# Autodesk Inventor assembly: Rear Z Axis
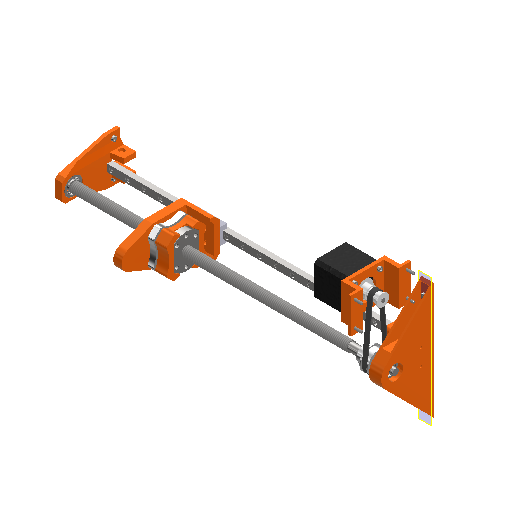
[picture p0: Inventor's stored thumbnail of the model, 512x512]
Saved by Autodesk Inventor 2023.2 (Build 272271000, 271)
## iProperties
Created: 2023-02-15
Part Number: Rear Z Axis
Document SubType Name: Assembly
Designer: remop
Author: remop
## Documents named in this file (20)
- C:\Users\remop\OneDrive\Documents\Inventor\3D Printers\LuEVO\Mk5_FullKinematic\Z Axis v2\Rear\Rear Z Axis.iam
- C:\Users\remop\OneDrive\Documents\Inventor\3D Printers\LuEVO\Mk5_FullKinematic\Z Axis v2\Drivetrain\MGNR9_300mm.ipt
- C:\Users\remop\OneDrive\Documents\Inventor\3D Printers\LuEVO\Mk5_FullKinematic\Z Axis v2\Drivetrain\MGN9H.ipt
- C:\Users\remop\OneDrive\Documents\Inventor\3D Printers\LuEVO\Mk5_FullKinematic\Z Axis v2\Rear\Rear Z Axis Top Bearing.ipt
- C:\Users\remop\OneDrive\Documents\Inventor\Content Center Files\R2023\en-US\AS 1420\AS 1420 - 1973 - M3 x 6.ipt
- C:\Users\remop\OneDrive\Documents\Inventor\Content Center Files\R2023\en-US\BS 290 SKF(21)\BS 290 SKF - SKF 608-RS1.ipt
- C:\Users\remop\OneDrive\Documents\Inventor\3D Printers\LuEVO\Mk5_FullKinematic\Z Axis v2\Drivetrain\Z Axis Ball Screw Bearing.ipt
- C:\Users\remop\OneDrive\Documents\Inventor\3D Printers\LuEVO\Mk5_FullKinematic\Z Axis v2\Drivetrain\Z Axis Ball Screw.ipt
- C:\Users\remop\OneDrive\Documents\Inventor\3D Printers\LuEVO\Mk5_FullKinematic\Z Axis v2\WobbleX WS12 Bottom.ipt
- C:\Users\remop\OneDrive\Documents\Inventor\3D Printers\LuEVO\Mk5_FullKinematic\Z Axis v2\WobbleX WS12.ipt
- C:\Users\remop\OneDrive\Documents\Inventor\3D Printers\LuEVO\Mk5_FullKinematic\Z Axis v2\Rear\Rear Z Axis Carriage.ipt
- C:\Users\remop\OneDrive\Documents\Inventor\3D Printers\LuEVO\Mk5_FullKinematic\Z Axis v2\Drivetrain\Z Axis Belt Pulley.ipt
- C:\Users\remop\OneDrive\Documents\Inventor\3D Printers\LuEVO\Mk5_FullKinematic\Z Axis v2\Rear\Rear Z Axis Bottom Bearing.ipt
- C:\Users\remop\OneDrive\Documents\Inventor\3D Printers\LuEVO\Mk5_FullKinematic\Z Axis v2\Drivetrain\Z Axis Belt.ipt
- C:\Users\remop\OneDrive\Documents\Inventor\3D Printers\LuEVO\Mk5_FullKinematic\Z Axis v2\Drivetrain\Z Axis Motor (Stepper).ipt
- C:\Users\remop\OneDrive\Documents\Inventor\3D Printers\LuEVO\Mk5_FullKinematic\XY Motion System\Belt Drives\Belt Pulley.ipt
- C:\Users\remop\OneDrive\Documents\Inventor\3D Printers\LuEVO\Mk5_FullKinematic\Z Axis v2\Drivetrain\Z Axis Motor Bracket.ipt
- C:\Users\remop\OneDrive\Documents\Inventor\Content Center Files\R2023\en-US\AS 1420\AS 1420 - 1973 - M3 x 8.ipt
- C:\Users\remop\OneDrive\Documents\Inventor\Content Center Files\R2023\en-US\AS 1420\AS 1420 - 1973 - M3 x 12.ipt
- C:\Users\remop\OneDrive\Documents\Inventor\Content Center Files\R2023\en-US\BS 1804\BS 1804-2 - 3 x 10.ipt
## Components (49 placed, 19 different names)
1. MGNR9_300mm:1 — Mate:1, Mate:2, Mate:3, Mate:4, Flush:1, Insert:4, Insert:7, Insert:8, Insert:9, Insert:10, Insert:11, Insert:12, Insert:13, Insert:14, Insert:15, Insert:16, Insert:17, Insert:18, Insert:19, Insert:20
2. MGN9H:1 — Mate:1, Mate:2, Angle:1, Flush:2, Rigid:4
3. Rear Z Axis Top Bearing:1 — Mate:3, Mate:4, Flush:1, Insert:1, Insert:2, Insert:3, Rigid:1
4. AS 1420 - Metric M3 x 6:1 — Insert:1
5. AS 1420 - Metric M3 x 6:2 — Insert:2
6. AS 1420 - Metric M3 x 6:3 — Insert:3
7. AS 1420 - Metric M3 x 6:4 — Insert:4
8. AS 1420 - Metric M3 x 6:7 — Insert:7
9. AS 1420 - Metric M3 x 6:8 — Insert:8
10. AS 1420 - Metric M3 x 6:9 — Insert:9
11. AS 1420 - Metric M3 x 6:10 — Insert:10
12. AS 1420 - Metric M3 x 6:11 — Insert:11
13. AS 1420 - Metric M3 x 6:12 — Insert:12
14. AS 1420 - Metric M3 x 6:13 — Insert:13
15. AS 1420 - Metric M3 x 6:14 — Insert:14
16. AS 1420 - Metric M3 x 6:15 — Insert:15
17. AS 1420 - Metric M3 x 6:16 — Insert:16
18. AS 1420 - Metric M3 x 6:17 — Insert:17
19. AS 1420 - Metric M3 x 6:18 — Insert:18
20. AS 1420 - Metric M3 x 6:19 — Insert:19
21. AS 1420 - Metric M3 x 6:20 — Insert:20
22. BS 290 SKF- with RS1 seal SKF 608-RS1:1 — Rigid:1, Rigid:2
23. BS 290 SKF- with RS1 seal SKF 608-RS1:2 — Rigid:6
24. Z Axis Ball Screw Bearing:1 — Cylindrical:1, Angle:1, Flush:2, Rotational:1, Mate:5
25. Z Axis Ball Screw:1 — Rigid:2, Cylindrical:1, Mate:5, Rigid:5, Rigid:6, Flush:3
26. WobbleX WS12 Bottom:1 — Rotational:1, Rigid:3
27. WobbleX WS12:1 — Rigid:3
28. Rear Z Axis Carriage:1 — Rigid:4, Rigid:8, Rigid:9, Rigid:10
29. Z Axis Belt Pulley:1 — Rigid:5, Rotational:2
30. Rear Z Axis Bottom Bearing:1 — Flush:3, Flush:4, Insert:25, Insert:26, Insert:27, Insert:28
31. Z Axis Belt:1 — Rotational:2, Rotational:3
32. Z Axis Motor (Stepper):1 — Rotational:3, Flush:4, Rotational:4, Rigid:7
33. Belt Pulley:1 — Rotational:4
34. Z Axis Motor Bracket:1 — Rigid:7, Insert:21, Insert:22, Insert:23, Insert:24, Insert:29, Insert:30, Insert:31, Insert:32
35. AS 1420 - Metric M3 x 8:1 — Insert:21
36. AS 1420 - Metric M3 x 8:2 — Insert:22
37. AS 1420 - Metric M3 x 8:3 — Insert:23
38. AS 1420 - Metric M3 x 8:4 — Insert:24
39. AS 1420 - Metric M3 x 6:21 — Insert:25
40. AS 1420 - Metric M3 x 6:22 — Insert:26
41. AS 1420 - Metric M3 x 6:23 — Insert:27
42. AS 1420 - Metric M3 x 6:24 — Insert:28
43. AS 1420 - Metric M3 x 12:1 — Insert:29
44. AS 1420 - Metric M3 x 12:2 — Insert:30
45. AS 1420 - Metric M3 x 12:3 — Insert:31
46. AS 1420 - Metric M3 x 12:4 — Insert:32
47. BS 1804 : Part 2 3 x 10:1 — Rigid:8
48. BS 1804 : Part 2 3 x 10:2 — Rigid:10
49. BS 1804 : Part 2 3 x 10:3 — Rigid:9
## Relationships (55: Insert 30, WeldJoint 10, Mate 5, Flush 4, RevoluteJoint 4, CylindricalJoint 1, Angle 1)
- Mate:1: MGNR9_300mm:1 ↔ MGN9H:1
- Mate:2: MGNR9_300mm:1 ↔ MGN9H:1
- Mate:3 (3 mm): MGNR9_300mm:1 ↔ Rear Z Axis Top Bearing:1
- Mate:4 (1 mm): MGNR9_300mm:1 ↔ Rear Z Axis Top Bearing:1
- Flush:1: MGNR9_300mm:1 ↔ Rear Z Axis Top Bearing:1
- Insert:1: Rear Z Axis Top Bearing:1 ↔ AS 1420 - Metric M3 x 6:1
- Insert:2: Rear Z Axis Top Bearing:1 ↔ AS 1420 - Metric M3 x 6:2
- Insert:3: Rear Z Axis Top Bearing:1 ↔ AS 1420 - Metric M3 x 6:3
- Insert:4: MGNR9_300mm:1 ↔ AS 1420 - Metric M3 x 6:4
- Insert:7: MGNR9_300mm:1 ↔ AS 1420 - Metric M3 x 6:7
- Insert:8: MGNR9_300mm:1 ↔ AS 1420 - Metric M3 x 6:8
- Insert:9: MGNR9_300mm:1 ↔ AS 1420 - Metric M3 x 6:9
- Insert:10: MGNR9_300mm:1 ↔ AS 1420 - Metric M3 x 6:10
- Insert:11: MGNR9_300mm:1 ↔ AS 1420 - Metric M3 x 6:11
- Insert:12: MGNR9_300mm:1 ↔ AS 1420 - Metric M3 x 6:12
- Insert:13: MGNR9_300mm:1 ↔ AS 1420 - Metric M3 x 6:13
- Insert:14: MGNR9_300mm:1 ↔ AS 1420 - Metric M3 x 6:14
- Insert:15: MGNR9_300mm:1 ↔ AS 1420 - Metric M3 x 6:15
- Insert:16: MGNR9_300mm:1 ↔ AS 1420 - Metric M3 x 6:16
- Insert:17: MGNR9_300mm:1 ↔ AS 1420 - Metric M3 x 6:17
- Insert:18: MGNR9_300mm:1 ↔ AS 1420 - Metric M3 x 6:18
- Insert:19: MGNR9_300mm:1 ↔ AS 1420 - Metric M3 x 6:19
- Insert:20: MGNR9_300mm:1 ↔ AS 1420 - Metric M3 x 6:20
- Rigid:1 [WeldJoint]: Rear Z Axis Top Bearing:1 ↔ BS 290 SKF- with RS1 seal SKF 608-RS1:1
- Rigid:2 [WeldJoint] (1 mm): BS 290 SKF- with RS1 seal SKF 608-RS1:1 ↔ Z Axis Ball Screw:1
- Cylindrical:1: Z Axis Ball Screw Bearing:1 ↔ Z Axis Ball Screw:1
- Angle:1 (0 deg): MGN9H:1 ↔ Z Axis Ball Screw Bearing:1
- Flush:2: MGN9H:1 ↔ Z Axis Ball Screw Bearing:1
- Rotational:1 [RevoluteJoint]: Z Axis Ball Screw Bearing:1 ↔ WobbleX WS12 Bottom:1
- Rigid:3 [WeldJoint] (-2 mm): WobbleX WS12 Bottom:1 ↔ WobbleX WS12:1
- Mate:5 (200 mm): Z Axis Ball Screw Bearing:1 ↔ Z Axis Ball Screw:1
- Rigid:4 [WeldJoint]: MGN9H:1 ↔ Rear Z Axis Carriage:1
- Rigid:5 [WeldJoint] (-5 mm): Z Axis Ball Screw:1 ↔ Z Axis Belt Pulley:1
- Rigid:6 [WeldJoint]: BS 290 SKF- with RS1 seal SKF 608-RS1:2 ↔ Z Axis Ball Screw:1
- Flush:3: Z Axis Ball Screw:1 ↔ Rear Z Axis Bottom Bearing:1
- Rotational:2 [RevoluteJoint]: Z Axis Belt Pulley:1 ↔ Z Axis Belt:1
- Rotational:3 [RevoluteJoint] (-16.35 mm): Z Axis Belt:1 ↔ Z Axis Motor (Stepper):1
- Flush:4 (25 mm): Rear Z Axis Bottom Bearing:1 ↔ Z Axis Motor (Stepper):1
- Rotational:4 [RevoluteJoint] (-0.5 mm): Z Axis Motor (Stepper):1 ↔ Belt Pulley:1
- Rigid:7 [WeldJoint]: Z Axis Motor (Stepper):1 ↔ Z Axis Motor Bracket:1
- Insert:21: Z Axis Motor Bracket:1 ↔ AS 1420 - Metric M3 x 8:1
- Insert:22: Z Axis Motor Bracket:1 ↔ AS 1420 - Metric M3 x 8:2
- Insert:23: Z Axis Motor Bracket:1 ↔ AS 1420 - Metric M3 x 8:3
- Insert:24: Z Axis Motor Bracket:1 ↔ AS 1420 - Metric M3 x 8:4
- Insert:25: Rear Z Axis Bottom Bearing:1 ↔ AS 1420 - Metric M3 x 6:21
- Insert:26: Rear Z Axis Bottom Bearing:1 ↔ AS 1420 - Metric M3 x 6:22
- Insert:27: Rear Z Axis Bottom Bearing:1 ↔ AS 1420 - Metric M3 x 6:23
- Insert:28: Rear Z Axis Bottom Bearing:1 ↔ AS 1420 - Metric M3 x 6:24
- Insert:29: Z Axis Motor Bracket:1 ↔ AS 1420 - Metric M3 x 12:1
- Insert:30: Z Axis Motor Bracket:1 ↔ AS 1420 - Metric M3 x 12:2
- Insert:31: Z Axis Motor Bracket:1 ↔ AS 1420 - Metric M3 x 12:3
- Insert:32: Z Axis Motor Bracket:1 ↔ AS 1420 - Metric M3 x 12:4
- Rigid:8 [WeldJoint] (0.5 mm): Rear Z Axis Carriage:1 ↔ BS 1804 : Part 2 3 x 10:1
- Rigid:9 [WeldJoint] (0.5 mm): Rear Z Axis Carriage:1 ↔ BS 1804 : Part 2 3 x 10:3
- Rigid:10 [WeldJoint] (0.5 mm): Rear Z Axis Carriage:1 ↔ BS 1804 : Part 2 3 x 10:2
